# Autodesk Inventor assembly: Assembly_final
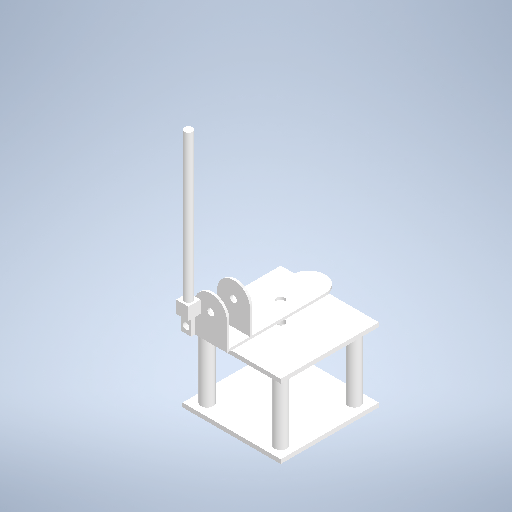
[picture p0: Inventor's stored thumbnail of the model, 512x512]
Saved by Autodesk Inventor 2025.3 (Build 293356000, 356)
## iProperties
Created: 2025-07-22
Part Number: Assembly_final
Document SubType Name: Assembly
Designer: KEVIN
Author: KEVIN
## Documents named in this file (4)
- C:\Users\KEVIN\OneDrive\Documentos\modern_control_project\inverted-pendulum\cad\Assembly_final.iam
- C:\Users\KEVIN\OneDrive\Documentos\modern_control_project\inverted-pendulum\cad\Base_engine.ipt
- C:\Users\KEVIN\OneDrive\Documentos\modern_control_project\inverted-pendulum\cad\Central_base.ipt
- C:\Users\KEVIN\OneDrive\Documentos\modern_control_project\inverted-pendulum\cad\pendulum.ipt
## Components (3 placed, 3 different names)
1. Base_engine:1 — Coincidencia:1, Coincidencia:2
2. Central_base:1 — Coincidencia:2
3. pendulum:1 — Coincidencia:1
## Relationships (2: Mate 2)
- Coincidencia:1 [Mate]: Base_engine:1 ↔ pendulum:1
- Coincidencia:2 [Mate]: Base_engine:1 ↔ Central_base:1
